# Autodesk Inventor assembly: Card Cage
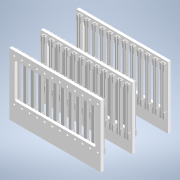
[picture p0: Inventor's stored thumbnail of the model, 180x180]
Saved by Autodesk Inventor 2021 (Build 250183000, 183)
## iProperties
Created: 2022-07-24
Part Number: Card Cage
Document SubType Name: Assembly
Designer: erics
Author: erics
## Documents named in this file (3)
- D:\Users\erics\Documents\16B\Mechanical\Card Cage.iam
- D:\Users\erics\Documents\16B\Mechanical\Center Wall.ipt
- D:\Users\erics\Documents\16B\Mechanical\CCA Rail.ipt
## Components (51 placed, 2 different names)
1. Center Wall:1 — Insert:1, Insert:2, Insert:3, Insert:4, Mate:1, Mate:2, Mate:3, Flush:1, Flush:2, Flush:3, Flush:4, Flush:5, Flush:6
2. Center Wall:2 — Flush:1, Flush:2, Flush:3, Insert:5, Insert:6
3. Center Wall:3 — Flush:4, Flush:5, Flush:6, Insert:7, Insert:8
4. CCA Rail:4 — Insert:7, Insert:8
5. CCA Rail:2 — Insert:3, Insert:4
6. CCA Rail:1 — Insert:1, Insert:2
7. CCA Rail:3 — Insert:5, Insert:6
8. CCA Rail:5
9. CCA Rail:6
10. CCA Rail:7
11. CCA Rail:8
12. CCA Rail:9
13. CCA Rail:10
14. CCA Rail:11
15. CCA Rail:12
16. CCA Rail:13
17. CCA Rail:14
18. CCA Rail:15
19. CCA Rail:16
20. CCA Rail:17
21. CCA Rail:18
22. CCA Rail:19
23. CCA Rail:20
24. CCA Rail:21
25. CCA Rail:22
26. CCA Rail:23
27. CCA Rail:24
28. CCA Rail:25
29. CCA Rail:26
30. CCA Rail:27
31. CCA Rail:28
32. CCA Rail:29
33. CCA Rail:30
34. CCA Rail:31
35. CCA Rail:32
36. CCA Rail:33
37. CCA Rail:34
38. CCA Rail:35
39. CCA Rail:36
40. CCA Rail:37
41. CCA Rail:38
42. CCA Rail:39
43. CCA Rail:40
44. CCA Rail:41
45. CCA Rail:42
46. CCA Rail:43
47. CCA Rail:44
48. CCA Rail:45
49. CCA Rail:46
50. CCA Rail:47
51. CCA Rail:48
## Component patterns: (12 elements, first: CCA Rail:4 + CCA Rail:2 + CCA Rail:1 + CCA Rail:3)
## Relationships (17: Insert 8, Flush 6, Mate 3)
- Insert:1: Center Wall:1 ↔ CCA Rail:1
- Insert:2: Center Wall:1 ↔ CCA Rail:1
- Insert:3: Center Wall:1 ↔ CCA Rail:2
- Insert:4: Center Wall:1 ↔ CCA Rail:2
- Mate:1: Center Wall:1
- Mate:2: Center Wall:1
- Mate:3: Center Wall:1
- Flush:1: Center Wall:1 ↔ Center Wall:2
- Flush:2: Center Wall:1 ↔ Center Wall:2
- Flush:3 (73.66 mm): Center Wall:1 ↔ Center Wall:2
- Flush:4: Center Wall:1 ↔ Center Wall:3
- Flush:5: Center Wall:1 ↔ Center Wall:3
- Flush:6 (83.82 mm): Center Wall:1 ↔ Center Wall:3
- Insert:5: Center Wall:2 ↔ CCA Rail:3
- Insert:6: Center Wall:2 ↔ CCA Rail:3
- Insert:7: Center Wall:3 ↔ CCA Rail:4
- Insert:8: Center Wall:3 ↔ CCA Rail:4
